# Autodesk Inventor assembly: 15102898-16-A-0300
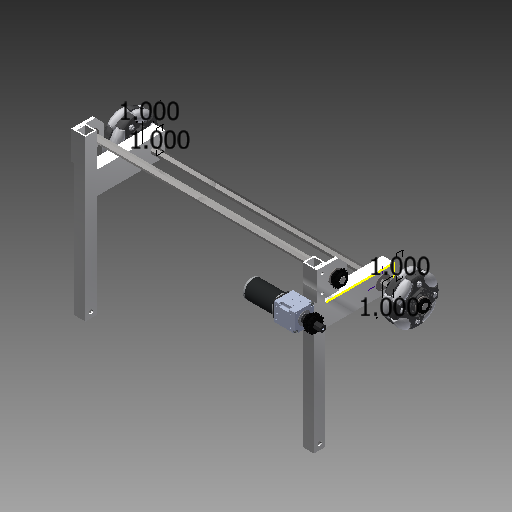
[picture p0: Inventor's stored thumbnail of the model, 512x512]
Saved by Autodesk Inventor 2017 (Build 210142000, 142)
## iProperties
Created: 2016-10-02
Part Number: 15102898-16-A-0300
Document SubType Name: Assembly
Designer: gus
Author: gus
## Documents named in this file (11)
- \\Mac\Home\Desktop\bunnybots 2016\15102898-16-Bunnybot-CAD\Bunnybot-To_be_renamed\15102898-16-A-0000\15102898-16-A-0300\15102898-16-A-0300.iam
- \\Mac\Home\Desktop\bunnybots 2016\15102898-16-Bunnybot-CAD\Bunnybot-To_be_renamed\15102898-16-A-0000\15102898-16-A-0300\15102898-16-P-0301.ipt
- \\Mac\Home\Desktop\bunnybots 2016\15102898-16-Bunnybot-CAD\Bunnybot-To_be_renamed\15102898-16-A-0000\15102898-16-A-0300\15102898-16-P-0302.ipt
- \\Mac\Home\Desktop\bunnybots 2016\15102898-16-Bunnybot-CAD\Bunnybot-To_be_renamed\15102898-16-A-0000\15102898-16-A-0300\Imported Components\217-3875-STEP-20140818.ipt
- \\Mac\Home\Desktop\bunnybots 2016\15102898-16-Bunnybot-CAD\Bunnybot-To_be_renamed\15102898-16-A-0000\15102898-16-A-0300\15102898-16-P-0303.ipt
- \\Mac\Home\Desktop\bunnybots 2016\15102898-16-Bunnybot-CAD\Bunnybot-To_be_renamed\15102898-16-A-0000\15102898-16-A-0300\Imported Components\217-2737.20121205.ipt
- \\Mac\Home\Desktop\bunnybots 2016\15102898-16-Bunnybot-CAD\Bunnybot-To_be_renamed\15102898-16-A-0000\15102898-16-A-0300\15102898-16-P-0304.ipt
- \\Mac\Home\Desktop\bunnybots 2016\15102898-16-Bunnybot-CAD\Bunnybot-To_be_renamed\15102898-16-A-0000\15102898-16-A-0300\Imported Components\am-3047_4inDuraOmniV2.ipt
- \\Mac\Home\Desktop\bunnybots 2016\15102898-16-Bunnybot-CAD\Bunnybot-To_be_renamed\15102898-16-A-0000\15102898-16-A-0300\15102898-16-P-0305.ipt
- \\Mac\Home\Desktop\bunnybots 2016\15102898-16-Bunnybot-CAD\Bunnybot-To_be_renamed\15102898-16-A-0000\15102898-16-A-0300\Imported Components\217-2642-STEP-20140807.ipt
- \\Mac\Home\Desktop\bunnybots 2016\15102898-16-Bunnybot-CAD\Bunnybot-To_be_renamed\15102898-16-A-0000\15102898-16-A-0300\Imported Components\BAG motor\VersaPlanetary-1-Stage-with-BAG-Motor.iam
## Components (28 placed, 10 different names)
1. 15102898-16-P-0301:1 — Flush:1, Flush:2, Mate:1, Flush:3, Flush:4, Mate:3, Mate:14, Flush:8, Flush:11, Mate:33, Flush:18
2. 15102898-16-P-0301:2 — Flush:1, Flush:2, Flush:5, Mate:2, Flush:6, Mate:3, Mate:15, Flush:14
3. 15102898-16-P-0302:1 — Mate:1, Flush:3, Flush:4, Cylindrical:1, Mate:5, Mate:38
4. 15102898-16-P-0302:2 — Flush:5, Mate:2, Flush:6, Cylindrical:2, Mate:4
5. 217-3875-STEP-20140818:1 — Cylindrical:2, Mate:4, Mate:13
6. 217-3875-STEP-20140818:2 — Cylindrical:1, Mate:5, Mate:6, Mate:7, Mate:34
7. 15102898-16-P-0303:1 — Mate:6, Mate:7, Mate:8, Mate:9, Mate:11, Mate:12, Flush:7, Mate:35, Mate:36
8. 217-2737.20121205:1 — Mate:11, Mate:12, Mate:13
9. 217-2737.20121205:2 — Mate:8, Mate:9, Flush:7, Mate:37
10. 15102898-16-P-0304:1 — Mate:14, Flush:8, Cylindrical:3, Mate:16, Flush:11, Flush:13
11. 15102898-16-P-0304:2 — Mate:15, Flush:13, Flush:14, Cylindrical:8, Mate:29
12. 217-3875-STEP-20140818:3 — Cylindrical:3, Mate:16, Mate:19, Mate:20, Mate:21
13. am-3047_4inDuraOmniV2:1 — Cylindrical:4, Mate:17, Mate:18, Cylindrical:5
14. 217-3875-STEP-20140818:4 — Cylindrical:4, Mate:17, Mate:21, Mate:39, Mate:40
15. 217-3875-STEP-20140818:5 — Mate:18, Cylindrical:5, Mate:25
16. 15102898-16-P-0305:1 — Mate:19, Mate:20, Flush:12, Mate:23, Mate:24, Mate:31, Mate:32, Mate:42, Mate:43
17. 217-2737.20121205:3 — Flush:12, Mate:23, Mate:24, Mate:25
18. 217-3875-STEP-20140818:6 — Cylindrical:8, Mate:29, Mate:30
19. am-3047_4inDuraOmniV2:2 — Cylindrical:7, Mate:28
20. 217-3875-STEP-20140818:7 — Flush:15, Flush:16, Flush:17, Mate:31
21. 217-2737.20121205:4 — Flush:16, Flush:17
22. 217-3875-STEP-20140818:8 — Cylindrical:7, Mate:28, Flush:15, Mate:30, Mate:32
23. 217-2642-STEP-20140807:1 — Cylindrical:9, Flush:19, Mate:44, Flush:20, Mate:45
24. 217-2642-STEP-20140807:2 — Mate:34, Mate:35, Mate:36, Mate:37, Flush:19, Rotation:1
25. 217-2642-STEP-20140807:3 — Mate:41, Mate:42, Mate:43
26. VersaPlanetary-1-Stage-with-BAG-Motor:1 [sub-assembly] — Mate:33, Flush:18, Cylindrical:9, Mate:38
27. 217-2737.20121205:5 — Mate:39, Mate:40, Mate:41
28. 217-2642-STEP-20140807:4 — Mate:44, Flush:20, Rotation:1, Mate:45
## Relationships (71: Mate 43, Flush 18, CylindricalJoint 9, RelateRotation 1)
- Flush:1: 15102898-16-P-0301:1 ↔ 15102898-16-P-0301:2
- Flush:2: 15102898-16-P-0301:1 ↔ 15102898-16-P-0301:2
- Mate:1: 15102898-16-P-0301:1 ↔ 15102898-16-P-0302:1
- Flush:3: 15102898-16-P-0301:1 ↔ 15102898-16-P-0302:1
- Flush:4: 15102898-16-P-0301:1 ↔ 15102898-16-P-0302:1
- Flush:5: 15102898-16-P-0301:2 ↔ 15102898-16-P-0302:2
- Mate:2: 15102898-16-P-0301:2 ↔ 15102898-16-P-0302:2
- Flush:6: 15102898-16-P-0301:2 ↔ 15102898-16-P-0302:2
- Mate:3 (482.6 mm): 15102898-16-P-0301:1 ↔ 15102898-16-P-0301:2
- Cylindrical:1: 15102898-16-P-0302:1 ↔ 217-3875-STEP-20140818:2
- Cylindrical:2: 15102898-16-P-0302:2 ↔ 217-3875-STEP-20140818:1
- Mate:4: 15102898-16-P-0302:2 ↔ 217-3875-STEP-20140818:1
- Mate:5: 15102898-16-P-0302:1 ↔ 217-3875-STEP-20140818:2
- Mate:6: 217-3875-STEP-20140818:2 ↔ 15102898-16-P-0303:1
- Mate:7: 217-3875-STEP-20140818:2 ↔ 15102898-16-P-0303:1
- Mate:8: 15102898-16-P-0303:1 ↔ 217-2737.20121205:2
- Mate:9: 15102898-16-P-0303:1 ↔ 217-2737.20121205:2
- Mate:11: 15102898-16-P-0303:1 ↔ 217-2737.20121205:1
- Mate:12: 15102898-16-P-0303:1 ↔ 217-2737.20121205:1
- Mate:13: 217-3875-STEP-20140818:1 ↔ 217-2737.20121205:1
- Flush:7: 15102898-16-P-0303:1 ↔ 217-2737.20121205:2
- Mate:14: 15102898-16-P-0301:1 ↔ 15102898-16-P-0304:1
- Flush:8: 15102898-16-P-0301:1 ↔ 15102898-16-P-0304:1
- Mate:15: 15102898-16-P-0301:2 ↔ 15102898-16-P-0304:2
- Cylindrical:3: 15102898-16-P-0304:1 ↔ 217-3875-STEP-20140818:3
- Mate:16: 15102898-16-P-0304:1 ↔ 217-3875-STEP-20140818:3
- Cylindrical:4: am-3047_4inDuraOmniV2:1 ↔ 217-3875-STEP-20140818:4
- Mate:17: am-3047_4inDuraOmniV2:1 ↔ 217-3875-STEP-20140818:4
- Mate:18: am-3047_4inDuraOmniV2:1 ↔ 217-3875-STEP-20140818:5
- Cylindrical:5: am-3047_4inDuraOmniV2:1 ↔ 217-3875-STEP-20140818:5
- Mate:19: 217-3875-STEP-20140818:3 ↔ 15102898-16-P-0305:1
- Mate:20: 217-3875-STEP-20140818:3 ↔ 15102898-16-P-0305:1
- Mate:21: 217-3875-STEP-20140818:3 ↔ 217-3875-STEP-20140818:4
- Flush:11 (76.2 mm): 15102898-16-P-0301:1 ↔ 15102898-16-P-0304:1
- Flush:12: 15102898-16-P-0305:1 ↔ 217-2737.20121205:3
- Mate:23: 15102898-16-P-0305:1 ↔ 217-2737.20121205:3
- Mate:24: 15102898-16-P-0305:1 ↔ 217-2737.20121205:3
- Mate:25: 217-3875-STEP-20140818:5 ↔ 217-2737.20121205:3
- Flush:13: 15102898-16-P-0304:1 ↔ 15102898-16-P-0304:2
- Flush:14: 15102898-16-P-0301:2 ↔ 15102898-16-P-0304:2
- [Mate]: am-3047_4inDuraOmniV2:2 ↔ 217-3875-STEP-20140818:7
- [CylindricalJoint]: am-3047_4inDuraOmniV2:2 ↔ 217-3875-STEP-20140818:7
- [Mate]: 217-3875-STEP-20140818:7 ↔ 217-2737.20121205:4
- Cylindrical:7: am-3047_4inDuraOmniV2:2 ↔ 217-3875-STEP-20140818:8
- Mate:28: am-3047_4inDuraOmniV2:2 ↔ 217-3875-STEP-20140818:8
- Flush:15: 217-3875-STEP-20140818:7 ↔ 217-3875-STEP-20140818:8
- Cylindrical:8: 15102898-16-P-0304:2 ↔ 217-3875-STEP-20140818:6
- Mate:29: 15102898-16-P-0304:2 ↔ 217-3875-STEP-20140818:6
- Mate:30: 217-3875-STEP-20140818:6 ↔ 217-3875-STEP-20140818:8
- Flush:16: 217-3875-STEP-20140818:7 ↔ 217-2737.20121205:4
- Flush:17: 217-3875-STEP-20140818:7 ↔ 217-2737.20121205:4
- Mate:31: 15102898-16-P-0305:1 ↔ 217-3875-STEP-20140818:7
- Mate:32: 15102898-16-P-0305:1 ↔ 217-3875-STEP-20140818:8
- Mate:33: 15102898-16-P-0301:1 ↔ VersaPlanetary-1-Stage-with-BAG-Motor:1
- Flush:18: 15102898-16-P-0301:1 ↔ VersaPlanetary-1-Stage-with-BAG-Motor:1
- Mate:34: 217-3875-STEP-20140818:2 ↔ 217-2642-STEP-20140807:2
- Mate:35: 15102898-16-P-0303:1 ↔ 217-2642-STEP-20140807:2
- Mate:36: 15102898-16-P-0303:1 ↔ 217-2642-STEP-20140807:2
- Mate:37: 217-2737.20121205:2 ↔ 217-2642-STEP-20140807:2
- Cylindrical:9: 217-2642-STEP-20140807:1 ↔ VersaPlanetary-1-Stage-with-BAG-Motor:1
- Mate:38: 15102898-16-P-0302:1 ↔ VersaPlanetary-1-Stage-with-BAG-Motor:1
- Mate:39: 217-3875-STEP-20140818:4 ↔ 217-2737.20121205:5
- Mate:40: 217-3875-STEP-20140818:4 ↔ 217-2737.20121205:5
- Mate:41: 217-2642-STEP-20140807:3 ↔ 217-2737.20121205:5
- Mate:42: 15102898-16-P-0305:1 ↔ 217-2642-STEP-20140807:3
- Mate:43: 15102898-16-P-0305:1 ↔ 217-2642-STEP-20140807:3
- Flush:19: 217-2642-STEP-20140807:1 ↔ 217-2642-STEP-20140807:2
- Mate:44: 217-2642-STEP-20140807:1 ↔ 217-2642-STEP-20140807:4
- Flush:20: 217-2642-STEP-20140807:1 ↔ 217-2642-STEP-20140807:4
- Rotation:1 [RelateRotation] (1 ul): 217-2642-STEP-20140807:2 ↔ 217-2642-STEP-20140807:4
- Mate:45: 217-2642-STEP-20140807:1 ↔ 217-2642-STEP-20140807:4
## Named parameters: d49_d46 = 0 mm, d50_d35 = 0 mm, d51_d36 = -49.171591 deg, d52_d37 = 0.9585 mm
